# Autodesk Inventor assembly: backmotors
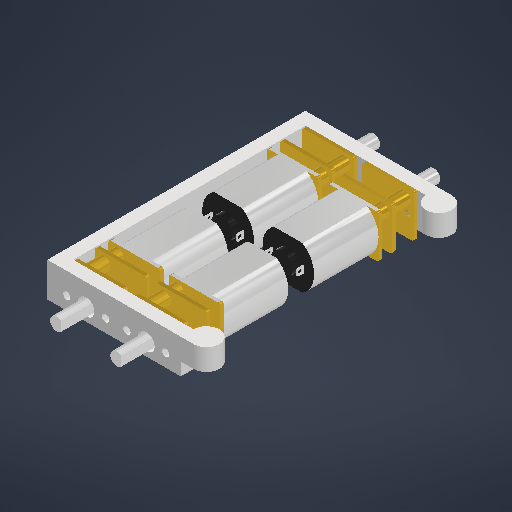
[picture p0: Inventor's stored thumbnail of the model, 512x512]
Saved by Autodesk Inventor 2026.2 (Build 302298010, 298A)
## iProperties
Created: 2026-04-27
Part Number: backmotors
Document SubType Name: Assembly
Designer: karol
Author: karol
## Documents named in this file (3)
- C:\Users\karol\OneDrive\Dokumenty\GitHub\bolt\bolt\cad\assembly\backmotors.iam
- C:\Users\karol\OneDrive\Dokumenty\GitHub\bolt\bolt\cad\ready parts\bmw.ipt
- C:\Users\karol\OneDrive\Dokumenty\GitHub\bolt\bolt\cad\ready parts\Pololu #2218 Micro Metal Gearmotor HP.ipt
## Components (5 placed, 2 different names)
1. bmw:1 — Mate:1, Mate:2, Mate:3, Mate:4, Mate:5, Mate:6, Mate:7, Mate:8, Mate:9, Mate:10, Mate:11, Mate:12, Mate:13, Mate:14
2. Pololu #2218 Micro Metal Gearmotor HP:1 — Mate:5, Mate:6, Mate:12
3. Pololu #2218 Micro Metal Gearmotor HP:2 — Mate:7, Mate:8, Mate:11, Mate:13
4. Pololu #2218 Micro Metal Gearmotor HP:3 — Mate:3, Mate:4, Mate:9
5. Pololu #2218 Micro Metal Gearmotor HP:4 — Mate:1, Mate:2, Mate:10, Mate:14
## Relationships (14: Mate 14)
- Mate:1: bmw:1 ↔ Pololu #2218 Micro Metal Gearmotor HP:4
- Mate:2: bmw:1 ↔ Pololu #2218 Micro Metal Gearmotor HP:4
- Mate:3: bmw:1 ↔ Pololu #2218 Micro Metal Gearmotor HP:3
- Mate:4: bmw:1 ↔ Pololu #2218 Micro Metal Gearmotor HP:3
- Mate:5: bmw:1 ↔ Pololu #2218 Micro Metal Gearmotor HP:1
- Mate:6: bmw:1 ↔ Pololu #2218 Micro Metal Gearmotor HP:1
- Mate:7: bmw:1 ↔ Pololu #2218 Micro Metal Gearmotor HP:2
- Mate:8: bmw:1 ↔ Pololu #2218 Micro Metal Gearmotor HP:2
- Mate:9: bmw:1 ↔ Pololu #2218 Micro Metal Gearmotor HP:3
- Mate:10: bmw:1 ↔ Pololu #2218 Micro Metal Gearmotor HP:4
- Mate:11: bmw:1 ↔ Pololu #2218 Micro Metal Gearmotor HP:2
- Mate:12: bmw:1 ↔ Pololu #2218 Micro Metal Gearmotor HP:1
- Mate:13: bmw:1 ↔ Pololu #2218 Micro Metal Gearmotor HP:2
- Mate:14: bmw:1 ↔ Pololu #2218 Micro Metal Gearmotor HP:4
